# Autodesk Inventor assembly: Plataforma_giratoria_4p
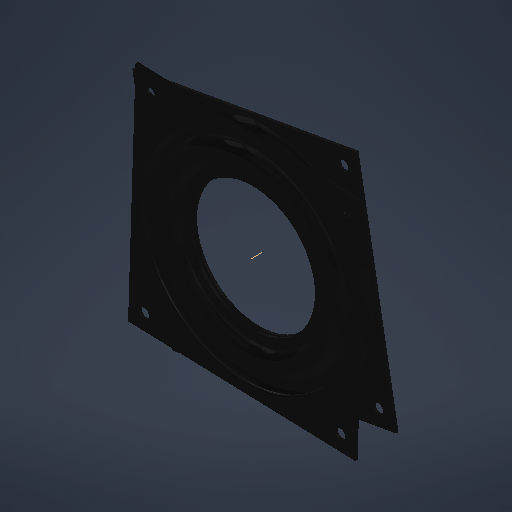
[picture p0: Inventor's stored thumbnail of the model, 512x512]
Saved by Autodesk Inventor 2025.2 (Build 292293000, 293)
## iProperties
Created: 2025-04-27
Part Number: Plataforma_giratoria_4p
Document SubType Name: Assembly
Designer: Tiago
Author: Tiago
## Documents named in this file (3)
- C:\Users\Tiago\Documents\Inventor\Exp. Braço v1\Plataforma_giratoria_4p.iam
- C:\Users\Tiago\Documents\Inventor\Exp. Braço v1\plataforma_giratória_94L)4polegadas).ipt
- C:\Users\Tiago\Documents\Inventor\Exp. Braço v1\Plataforma_giratória_esfera.ipt
## Components (3 placed, 2 different names)
1. plataforma_giratória_94L)4polegadas):1 — Mate:1, Mate:2, Flush:1, Symmetry:1, Mate:3, Mate:4
2. plataforma_giratória_94L)4polegadas):2 — Mate:1, Mate:2, Symmetry:1
3. Plataforma_giratória_esfera:1 — Mate:4, Flush:2
## Relationships (7: Mate 4, Flush 2, Symmetry 1)
- Mate:1 (6.8 mm): plataforma_giratória_94L)4polegadas):1 ↔ plataforma_giratória_94L)4polegadas):2
- Mate:2: plataforma_giratória_94L)4polegadas):1 ↔ plataforma_giratória_94L)4polegadas):2
- Flush:1: plataforma_giratória_94L)4polegadas):1
- Symmetry:1: plataforma_giratória_94L)4polegadas):1 ↔ plataforma_giratória_94L)4polegadas):2
- Mate:3: plataforma_giratória_94L)4polegadas):1
- Mate:4: plataforma_giratória_94L)4polegadas):1 ↔ Plataforma_giratória_esfera:1
- Flush:2: Plataforma_giratória_esfera:1
